# Autodesk Inventor assembly: xzrailassembly
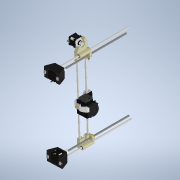
[picture p0: Inventor's stored thumbnail of the model, 180x180]
Saved by Autodesk Inventor 2020.2 (Build 242310000, 310)
## iProperties
Created: 2020-07-30
Part Number: xzrailassembly
Document SubType Name: Assembly
Designer: JK
Author: JK
## Documents named in this file (4)
- C:\Users\JK\Documents\Inventor\Anet Upgrade\xzrailassembly.iam
- C:\Users\JK\Documents\Inventor\Anet Upgrade\assemblyxrail.iam
- C:\Users\JK\Documents\Inventor\Anet Upgrade\8x380axis.ipt
- C:\Users\JK\Documents\Inventor\Anet Upgrade\ZMotorassembly.iam
## Components (5 placed, 3 different names)
1. assemblyxrail:1 [sub-assembly] — Mate:19, Mate:20, Mate:28, Angle:1, Angle:2
2. Wał:1 — Mate:19, Flush:5
3. Wał:2 — Mate:20, Flush:5
4. ZMotorassembly:1 [sub-assembly] — Angle:1, Flush:6
5. ZMotorassembly:2 [sub-assembly] — Mate:28, Angle:2, Flush:6
## Relationships (9: Mate 5, Flush 2, Angle 2)
- [Mate]: assemblyxrail:1 ↔ ZMotorassembly:1
- Mate:19: assemblyxrail:1 ↔ Wał:1
- Mate:20: assemblyxrail:1 ↔ Wał:2
- Flush:5: Wał:1 ↔ Wał:2
- [Mate]: Wał:1 ↔ ZMotorassembly:1
- Mate:28: assemblyxrail:1 ↔ ZMotorassembly:2
- Angle:1 (0 deg): assemblyxrail:1 ↔ ZMotorassembly:1
- Angle:2 (0 deg): assemblyxrail:1 ↔ ZMotorassembly:2
- Flush:6: ZMotorassembly:1 ↔ ZMotorassembly:2
